# Autodesk Inventor assembly: beercart assembly - mekatronik
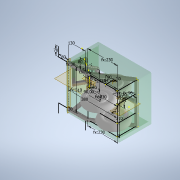
[picture p0: Inventor's stored thumbnail of the model, 180x180]
Saved by Autodesk Inventor 2022.2 (Build 262287000, 287)
## iProperties
_SolveAssemblyDoc: Frame Generator Solve Assembly
_Version: 15.0.0
Created: 2022-03-11
Part Number: beercart assembly - mekatronik
Document SubType Name: Assembly
Designer: foriw
Mass: 11477.2 g
Surface Area: 14355.3 cm^2
Volume: 8635.48 cm^3
Density: 1.32908 g/cm^3
Author: foriw
## Documents named in this file (9)
- H:\inventor ting\Mekatronik beercart git\Beercart CAD\Workspaces\Workspace\beercart assembly - mekatronik.iam
- H:\inventor ting\Mekatronik beercart git\Beercart CAD\Workspaces\Workspace\beercart- framwork - baseSketch.ipt
- H:\inventor ting\Mekatronik beercart git\Beercart CAD\Workspaces\Workspace\beercart assembly - mekatronik\Frame\Frame 1647030135921.iam
- H:\inventor ting\Mekatronik beercart git\Beercart CAD\Workspaces\Workspace\motor at24v.ipt
- H:\inventor ting\Mekatronik beercart git\Beercart CAD\Workspaces\Workspace\beer crate.ipt
- H:\inventor ting\Mekatronik beercart git\Beercart CAD\Workspaces\Workspace\Mekatronik-beerCart\frontwheel frame.ipt
- H:\inventor ting\Mekatronik beercart git\Beercart CAD\Workspaces\Workspace\motor at24v_MIR.ipt
- H:\inventor ting\Mekatronik beercart git\Beercart CAD\Workspaces\Workspace\FreeBackWheel.ipt
- H:\inventor ting\Mekatronik beercart git\Beercart CAD\Libraries\Content Center Files\en-US\ANSI B18.2.4.4M\ANSI B18.2.4.4M - M8 x 1,25.ipt
## Components (8 placed, 8 different names)
1. beercart- framwork - baseSketch:1
2. Frame 1647030135921:1 [sub-assembly] — Flush:3, Insert:2, Insert:3, Mate:2, Insert:4, Mate:3
3. motor at24v:1
4. beer crate:1 — Flush:2, Flush:3
5. frontwheel frame:1
6. motor at24v_MIR:1 — Insert:2, Insert:3, Mate:1
7. FreeBackWheel:1 — Mate:1, Mate:2, Mate:3
8. Metric Hex Flange Nuts - Metric M8 x 1,25:1 — Insert:4
## Relationships (9: Insert 4, Mate 3, Flush 2)
- Flush:2: beer crate:1
- Flush:3: Frame 1647030135921:1 ↔ beer crate:1
- [Insert]: Frame 1647030135921:1 ↔ motor at24v_MIR:1
- Insert:2: Frame 1647030135921:1 ↔ motor at24v_MIR:1
- Insert:3: Frame 1647030135921:1 ↔ motor at24v_MIR:1
- Mate:1: motor at24v_MIR:1 ↔ FreeBackWheel:1
- Mate:2 (0.5 mm): Frame 1647030135921:1 ↔ FreeBackWheel:1
- Insert:4: Frame 1647030135921:1 ↔ Metric Hex Flange Nuts - Metric M8 x 1,25:1
- Mate:3 (0.5 mm): Frame 1647030135921:1 ↔ FreeBackWheel:1
